# Autodesk Inventor assembly: MCbeamadj
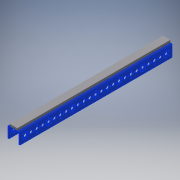
[picture p0: Inventor's stored thumbnail of the model, 180x180]
Saved by Autodesk Inventor 2016 (Build 200138000, 138)
## iProperties
Created: 2015-09-04
Part Number: MCbeamadj
Document SubType Name: Assembly
Designer: Tim
Author: Tim
## Documents named in this file (3)
- C:\Users\Tim\Documents\GitHub\phi_robotics\3d-models\FTC_Tetrix_KOP_Block_Party\Tim Bloot Designs\MCbeamadj.iam
- C:\Users\Tim\Documents\GitHub\phi_robotics\3d-models\FTC_Tetrix_KOP_Block_Party\Tim Bloot Designs\MCbeam.ipt
- C:\Users\Tim\Documents\GitHub\phi_robotics\3d-models\FTC_Tetrix_KOP_Block_Party\Tetrix_Kit_FTC\Autodesk Inventor Files\tetrix_c_channel-5.ipt
## Components (2 placed, 2 different names)
1. MCbeam:2 — Flush:1, Mate:1
2. tetrix_c_channel-5:1 — Flush:1, Mate:1
## Relationships (2: Flush 1, Mate 1)
- Flush:1: MCbeam:2 ↔ tetrix_c_channel-5:1
- Mate:1: MCbeam:2 ↔ tetrix_c_channel-5:1
